# Autodesk Inventor assembly: Assembly1
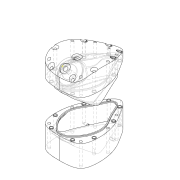
[picture p0: Inventor's stored thumbnail of the model, 180x180]
Saved by Autodesk Inventor 2018 (Build 220112000, 112)
## iProperties
Created: 2020-04-08
Part Number: Assembly1
Document SubType Name: Assembly
Designer: Matt
Author: Matt
## Documents named in this file (5)
- C:\Users\Matt\n95\v4\Assembly1.iam
- C:\Users\Matt\n95\v3\maskBodySolidV2.ipt
- C:\Users\Matt\n95\v4\moldLower.ipt
- C:\Users\Matt\n95\v4\maskBodySolidV2InnerTool.ipt
- C:\Users\Matt\n95\v4\moldUpper2.ipt
## Components (4 placed, 4 different names)
1. maskBodySolidV2:1 — Flush:2, Flush:3, Flush:4
2. moldLower:1 — Flush:1, Flush:5, Flush:6, Flush:7
3. maskBodySolidV2InnerTool:1 — Flush:2, Flush:3, Flush:4
4. moldUpper2:1 — Flush:5, Flush:6, Flush:7
## Relationships (7: Flush 7)
- Flush:1: moldLower:1
- Flush:2: maskBodySolidV2:1 ↔ maskBodySolidV2InnerTool:1
- Flush:3: maskBodySolidV2:1 ↔ maskBodySolidV2InnerTool:1
- Flush:4: maskBodySolidV2:1 ↔ maskBodySolidV2InnerTool:1
- Flush:5: moldLower:1 ↔ moldUpper2:1
- Flush:6: moldLower:1 ↔ moldUpper2:1
- Flush:7: moldLower:1 ↔ moldUpper2:1
